# Autodesk Inventor assembly: Assembly1
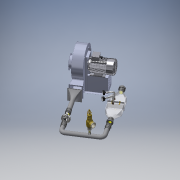
[picture p0: Inventor's stored thumbnail of the model, 180x180]
Saved by Autodesk Inventor 2017 (Build 210142000, 142)
## iProperties
Created: 2017-02-09
Part Number: Assembly1
Document SubType Name: Assembly
Designer: XuZhiqing
Author: XuZhiqing
## Documents named in this file (9)
- C:\Users\XuZhiqing\Desktop\Project01-CFD_the_sys\CAD-Whole Sys v1.02\ZSYSTEM\Assembly1.iam
- C:\Users\XuZhiqing\Desktop\Project01-CFD_the_sys\CAD-Whole Sys v1.02\safety relief valve\SRV.ipt
- C:\Users\XuZhiqing\Desktop\Project01-CFD_the_sys\CAD-Whole Sys v1.02\filter and gauge\filter and gauge\filter and gauge.iam
- C:\Users\XuZhiqing\Desktop\Project01-CFD_the_sys\CAD-Whole Sys v1.02\butterfly valve\Butterfly-valve-DIN-11850-male-male-DN50-open.ipt
- C:\Users\XuZhiqing\Desktop\Project01-CFD_the_sys\CAD-Whole Sys v1.02\ZSYSTEM\blower.ipt
- C:\Users\XuZhiqing\Desktop\Project01-CFD_the_sys\CAD-Whole Sys v1.02\ZSYSTEM\connector1.ipt
- C:\Users\XuZhiqing\Desktop\Project01-CFD_the_sys\CAD-Whole Sys v1.02\other\banjo male cam.ipt
- C:\Users\XuZhiqing\Desktop\Project01-CFD_the_sys\CAD-Whole Sys v1.02\other\big bend.ipt
- C:\Users\XuZhiqing\Desktop\Project01-CFD_the_sys\CAD-Whole Sys v1.02\ZSYSTEM\connector2.ipt
## Components (10 placed, 8 different names)
1. SRV:2 — Mate:11
2. filter and gauge:1 [sub-assembly] — Angle:3, Angle:4, Mate:9
3. Butterfly-valve-DIN-11850-male-male-DN50-open:1 — Angle:1, Mate:1, Mate:8
4. blower:1 — Flush:1, Flush:2, Angle:1, Angle:2
5. connector1:1 — Flush:1, Flush:2, Mate:1, Mate:2, Mate:3
6. banjo male cam:1 — Mate:2, Mate:3
7. connector2:1 — Mate:4, Mate:5, Mate:6, Mate:7, Angle:2, Angle:4, Mate:10, Angle:5
8. banjo male cam:2 — Mate:4, Mate:5, Mate:8
9. banjo male cam:3 — Mate:6, Mate:7, Angle:3, Mate:9
10. big bend:1 — Mate:10, Angle:5, Mate:11
## Relationships (18: Mate 11, Angle 5, Flush 2)
- Flush:1: blower:1 ↔ connector1:1
- Flush:2: blower:1 ↔ connector1:1
- Angle:1 (0 deg): Butterfly-valve-DIN-11850-male-male-DN50-open:1 ↔ blower:1
- Mate:1: Butterfly-valve-DIN-11850-male-male-DN50-open:1 ↔ connector1:1
- Mate:2: connector1:1 ↔ banjo male cam:1
- Mate:3: connector1:1 ↔ banjo male cam:1
- Mate:4: connector2:1 ↔ banjo male cam:2
- Mate:5: connector2:1 ↔ banjo male cam:2
- Mate:6: connector2:1 ↔ banjo male cam:3
- Mate:7: connector2:1 ↔ banjo male cam:3
- Mate:8: Butterfly-valve-DIN-11850-male-male-DN50-open:1 ↔ banjo male cam:2
- Angle:2 (0 deg): blower:1 ↔ connector2:1
- Angle:3 (0 deg): filter and gauge:1 ↔ banjo male cam:3
- Angle:4 (180 deg): filter and gauge:1 ↔ connector2:1
- Mate:9: filter and gauge:1 ↔ banjo male cam:3
- Mate:10: connector2:1 ↔ big bend:1
- Angle:5 (90 deg): connector2:1 ↔ big bend:1
- Mate:11: SRV:2 ↔ big bend:1
